# Autodesk Inventor assembly: sap_mechanism
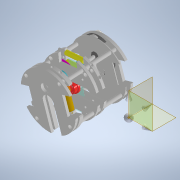
[picture p0: Inventor's stored thumbnail of the model, 180x180]
Saved by Autodesk Inventor 2021 (Build 250183000, 183)
## iProperties
Created: 2024-02-12
Part Number: sap_mechanism
Document SubType Name: Assembly
Designer: Sebastián
Author: Sebastián
## Documents named in this file (9)
- C:\Users\Sebastián\Documents\Inventor\PLD SAP\sap_mechanism.iam
- C:\Users\Sebastián\Documents\Inventor\PLD SAP\shaft_8mm.ipt
- C:\Users\Sebastián\Documents\Inventor\PLD SAP\modular\Design Accelerator\Worm Gears1.iam
- C:\Users\Sebastián\Documents\Inventor\PLD SAP\struct_shaft.ipt
- C:\Users\Sebastián\Documents\Inventor\PLD SAP\placa_2_3.iam
- C:\Users\Sebastián\Documents\Inventor\PLD SAP\170d_coupler.ipt
- C:\Users\Sebastián\Documents\Inventor\PLD SAP\placa_bottom.ipt
- C:\Users\Sebastián\Documents\Inventor\PLD SAP\rollers_plate.iam
- C:\Users\Sebastián\Documents\Inventor\PLD SAP\target_plate.iam
## Components (11 placed, 8 different names)
1. rollers_plate:1 [sub-assembly] — Cylindrical:8, Cylindrical:10, Cylindrical:11, Cylindrical:12, Tangent:1
2. target_plate:1 [sub-assembly] — Rotational:7, Rotational:8, Rotational:9, Rotational:10, Mate:1, Flush:1
3. Worm Gears:1 [sub-assembly] — Cylindrical:8, Cylindrical:9
4. shaft_8mm:3 — Cylindrical:9, Rigid:1
5. struct_shaft:1 — Rotational:8, Cylindrical:6
6. struct_shaft:2 — Rotational:9, Cylindrical:7, Cylindrical:11, Cylindrical:13
7. struct_shaft:3 — Rotational:10
8. struct_shaft:4 — Rotational:7
9. placa_2_3:1 [sub-assembly] — Cylindrical:6, Cylindrical:7, Mate:1, Cylindrical:10, Mate:2
10. 170d_coupler:1 — Rigid:1, Mate:2
11. placa_bottom:1 — Cylindrical:12, Cylindrical:13, Tangent:1, Flush:1
## Relationships (17: CylindricalJoint 8, RevoluteJoint 4, Mate 2, WeldJoint 1, Tangent 1, Flush 1)
- Rotational:7 [RevoluteJoint]: target_plate:1 ↔ struct_shaft:4
- Rotational:8 [RevoluteJoint]: target_plate:1 ↔ struct_shaft:1
- Rotational:9 [RevoluteJoint]: target_plate:1 ↔ struct_shaft:2
- Rotational:10 [RevoluteJoint]: target_plate:1 ↔ struct_shaft:3
- Cylindrical:6: struct_shaft:1 ↔ placa_2_3:1
- Cylindrical:7: struct_shaft:2 ↔ placa_2_3:1
- Mate:1 (1.5 mm): target_plate:1 ↔ placa_2_3:1
- Cylindrical:8: rollers_plate:1 ↔ Worm Gears:1
- Cylindrical:9: Worm Gears:1 ↔ shaft_8mm:3
- Cylindrical:10: rollers_plate:1 ↔ placa_2_3:1
- Cylindrical:11: rollers_plate:1 ↔ struct_shaft:2
- Rigid:1 [WeldJoint]: shaft_8mm:3 ↔ 170d_coupler:1
- Mate:2 (2 mm): placa_2_3:1 ↔ 170d_coupler:1
- Cylindrical:12: rollers_plate:1 ↔ placa_bottom:1
- Cylindrical:13: struct_shaft:2 ↔ placa_bottom:1
- Tangent:1: rollers_plate:1 ↔ placa_bottom:1
- Flush:1 (-140 mm): target_plate:1 ↔ placa_bottom:1
